# Autodesk Inventor assembly: DIFF_BARV2_ASM
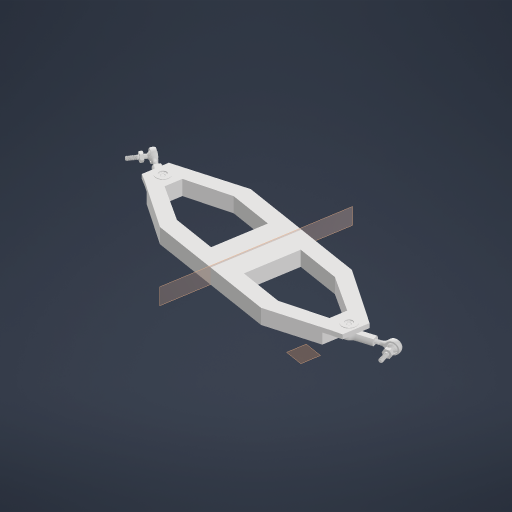
[picture p0: Inventor's stored thumbnail of the model, 512x512]
Saved by Autodesk Inventor 2023 (Build 270158000, 158)
## iProperties
Created: 2023-04-06
Part Number: DIFF_BARV2_ASM
Document SubType Name: Assembly
Designer: bugme
Author: bugme
## Documents named in this file (10)
- C:\Users\bugme\Desktop\Diff Bar\DIFF_BARV2_ASM.iam
- C:\Users\bugme\Desktop\Diff Bar\Diff_BarV2.ipt
- C:\Users\bugme\Desktop\Diff Bar\60645K211_Ball Joint Linkage.ipt
- C:\Users\bugme\Desktop\Diff Bar\59915K481_Corrosion-Resistant Ball Joint Rod End.ipt
- C:\Users\bugme\Desktop\Diff Bar\98381A505_Dowel Pin.ipt
- C:\Users\bugme\Desktop\Diff Bar\1293N114_Self-Aligning Flanged Ball Bearing.ipt
- C:\Users\bugme\Desktop\Diff Bar\1293N114_Self-Aligning Flanged Ball Bearing_MIR1.ipt
- C:\Users\bugme\Desktop\Diff Bar\59915K481_Corrosion-Resistant Ball Joint Rod End_MIR1.ipt
- C:\Users\bugme\Desktop\Diff Bar\60645K211_Ball Joint Linkage_MIR1.ipt
- C:\Users\bugme\Desktop\Diff Bar\98381A505_Dowel Pin_MIR1.ipt
## Components (9 placed, 9 different names)
1. Diff_BarV2:1 — Rotational:1, Mate:1, Angle:1, Rotational:5
2. 1293N114_Self-Aligning Flanged Ball Bearing:1 — Cylindrical:1, Rotational:1
3. 59915K481_Corrosion-Resistant Ball Joint Rod End:1 — Rotational:3, Cylindrical:3
4. 60645K211_Ball Joint Linkage:1 — Cylindrical:3
5. 98381A505_Dowel Pin:1 — Cylindrical:1, Rotational:3
6. 1293N114_Self-Aligning Flanged Ball Bearing_MIR1:1 — Cylindrical:5, Rotational:5
7. 59915K481_Corrosion-Resistant Ball Joint Rod End_MIR1:1 — Cylindrical:4, Rotational:4
8. 60645K211_Ball Joint Linkage_MIR1:1 — Cylindrical:4
9. 98381A505_Dowel Pin_MIR1:1 — Cylindrical:5, Rotational:4
## Relationships (10: CylindricalJoint 4, RevoluteJoint 4, Mate 1, Angle 1)
- Cylindrical:1: 1293N114_Self-Aligning Flanged Ball Bearing:1 ↔ 98381A505_Dowel Pin:1
- Rotational:1 [RevoluteJoint]: Diff_BarV2:1 ↔ 1293N114_Self-Aligning Flanged Ball Bearing:1
- Rotational:3 [RevoluteJoint]: 59915K481_Corrosion-Resistant Ball Joint Rod End:1 ↔ 98381A505_Dowel Pin:1
- Cylindrical:3: 59915K481_Corrosion-Resistant Ball Joint Rod End:1 ↔ 60645K211_Ball Joint Linkage:1
- Mate:1: Diff_BarV2:1
- Angle:1 (0 deg): Diff_BarV2:1
- Cylindrical:4: 59915K481_Corrosion-Resistant Ball Joint Rod End_MIR1:1 ↔ 60645K211_Ball Joint Linkage_MIR1:1
- Cylindrical:5: 1293N114_Self-Aligning Flanged Ball Bearing_MIR1:1 ↔ 98381A505_Dowel Pin_MIR1:1
- Rotational:4 [RevoluteJoint]: 59915K481_Corrosion-Resistant Ball Joint Rod End_MIR1:1 ↔ 98381A505_Dowel Pin_MIR1:1
- Rotational:5 [RevoluteJoint]: Diff_BarV2:1 ↔ 1293N114_Self-Aligning Flanged Ball Bearing_MIR1:1
